# Autodesk Inventor assembly: Assembly
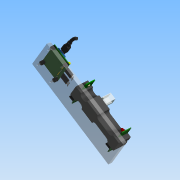
[picture p0: Inventor's stored thumbnail of the model, 180x180]
Saved by Autodesk Inventor 2016 (Build 200138000, 138)
## iProperties
Created: 2015-08-03
Part Number: Assembly
Document SubType Name: Assembly
Designer: Openlab
Author: Openlab
## Documents named in this file (8)
- D:\Alexey\HS-Spectrophotometer\parts\Luna\Assembly.iam
- D:\Alexey\HS-Spectrophotometer\parts\Luna\Luna_base.ipt
- D:\Alexey\HS-Spectrophotometer\parts\Common\Support_washer.ipt
- D:\Alexey\HS-Spectrophotometer\parts\Common\Microcontroller_board_Nano_square.iam
- D:\Alexey\HS-Spectrophotometer\parts\Luna\Luna_core.ipt
- D:\Alexey\HS-Spectrophotometer\parts\Test\LED_board.ipt
- D:\Alexey\HS-Spectrophotometer\parts\Test\Sensor_board.ipt
- D:\Alexey\HS-Spectrophotometer\parts\Common\Cuvette.ipt
## Components (10 placed, 7 different names)
1. Luna_base:1 — Mate:1, Mate:2, Mate:3, Mate:4, Mate:5, Mate:6, Mate:7, Mate:8, Mate:12, Flush:1, Flush:2
2. Support_washer:1 — Mate:1, Mate:5, Mate:9, Mate:11
3. Support_washer:2 — Mate:2, Mate:6
4. Support_washer:3 — Mate:3, Mate:7
5. Support_washer:4 — Mate:4, Mate:8, Mate:10
6. Microcontroller_board_Nano_square:1 [sub-assembly] — Mate:9, Mate:10, Mate:11
7. Luna_core:1 — Mate:12, Mate:13, Mate:14, Mate:15, Mate:16, Flush:1, Flush:2, Mate:17, Mate:18, Mate:19
8. LED_board:1 — Mate:13, Mate:14
9. Sensor_board:1 — Mate:15, Mate:16
10. Cuvette:1 — Mate:17, Mate:18, Mate:19
## Relationships (21: Mate 19, Flush 2)
- Mate:1: Luna_base:1 ↔ Support_washer:1
- Mate:2: Luna_base:1 ↔ Support_washer:2
- Mate:3: Luna_base:1 ↔ Support_washer:3
- Mate:4: Luna_base:1 ↔ Support_washer:4
- Mate:5: Luna_base:1 ↔ Support_washer:1
- Mate:6: Luna_base:1 ↔ Support_washer:2
- Mate:7: Luna_base:1 ↔ Support_washer:3
- Mate:8: Luna_base:1 ↔ Support_washer:4
- Mate:9: Support_washer:1 ↔ Microcontroller_board_Nano_square:1
- Mate:10: Support_washer:4 ↔ Microcontroller_board_Nano_square:1
- Mate:11: Support_washer:1 ↔ Microcontroller_board_Nano_square:1
- Mate:12: Luna_base:1 ↔ Luna_core:1
- Mate:13: Luna_core:1 ↔ LED_board:1
- Mate:14: Luna_core:1 ↔ LED_board:1
- Mate:15: Luna_core:1 ↔ Sensor_board:1
- Mate:16: Luna_core:1 ↔ Sensor_board:1
- Flush:1 (10 mm): Luna_base:1 ↔ Luna_core:1
- Flush:2 (20 mm): Luna_base:1 ↔ Luna_core:1
- Mate:17: Luna_core:1 ↔ Cuvette:1
- Mate:18: Luna_core:1 ↔ Cuvette:1
- Mate:19: Luna_core:1 ↔ Cuvette:1
